# Autodesk Inventor assembly: chain(e)
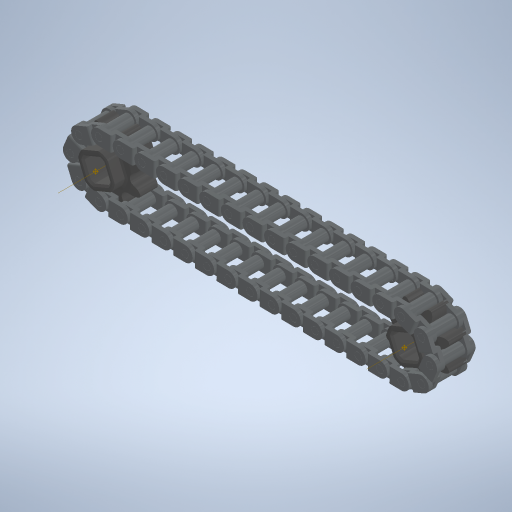
[picture p0: Inventor's stored thumbnail of the model, 512x512]
Saved by Autodesk Inventor 2023 (Build 270158000, 158)
## iProperties
Created: 2022-08-09
Part Number: chain(e)
Document SubType Name: Assembly
Designer: aaron
Author: aaron
## Documents named in this file (3)
- C:\Users\aaron\Documents\Inventor\Spin Up\library\Motion\New Sprockets\chain(e).iam
- C:\Users\aaron\Documents\Inventor\Spin Up\library\Motion\New Sprockets\8T.ipt
- C:\Users\aaron\Documents\Inventor\Spin Up\library\Motion\New Sprockets\IQ chain.ipt
## Components (38 placed, 2 different names)
1. 8T:1 — Mate:1, Mate:68, Mate:69, Mate:70, Mate:71, Flush:62, Mate:73
2. 8T:2 — Mate:1, Mate:63, Mate:64, Mate:65, Mate:66, Mate:67
3. IQ chain:12 — Mate:72, Mate:73
4. IQ chain:13
5. IQ chain:14
6. IQ chain:15
7. IQ chain:16 — Mate:31, Flush:30
8. IQ chain:17 — Mate:31, Flush:30
9. IQ chain:18
10. IQ chain:19
11. IQ chain:20
12. IQ chain:21
13. IQ chain:22
14. IQ chain:23
15. IQ chain:24
16. IQ chain:25
17. IQ chain:26 — Mate:63
18. IQ chain:27 — Mate:64
19. IQ chain:28 — Mate:65
20. IQ chain:29 — Mate:66
21. IQ chain:30 — Mate:67
22. IQ chain:31 — Mate:62, Flush:61
23. IQ chain:32 — Mate:62, Flush:61
24. IQ chain:33
25. IQ chain:34
26. IQ chain:35
27. IQ chain:36
28. IQ chain:37
29. IQ chain:38
30. IQ chain:39
31. IQ chain:40
32. IQ chain:41
33. IQ chain:42
34. IQ chain:43
35. IQ chain:44 — Mate:68
36. IQ chain:45 — Mate:69
37. IQ chain:46 — Mate:70
38. IQ chain:47 — Mate:71, Mate:72, Flush:62
## Relationships (83: Mate 47, Flush 36)
- Mate:1 (88.9 mm): 8T:1 ↔ 8T:2
- [Mate]: IQ chain:13 ↔ IQ chain:14
- [Flush]: IQ chain:13 ↔ IQ chain:14
- [Mate]: IQ chain:15 ↔ IQ chain:16
- [Flush]: IQ chain:15 ↔ IQ chain:16
- [Mate]: IQ chain:14 ↔ IQ chain:15
- [Flush]: IQ chain:14 ↔ IQ chain:15
- [Mate]: IQ chain:12 ↔ IQ chain:13
- [Flush]: IQ chain:12 ↔ IQ chain:13
- [Mate]: IQ chain:18 ↔ IQ chain:19
- [Flush]: IQ chain:18 ↔ IQ chain:19
- [Mate]: IQ chain:17 ↔ IQ chain:18
- [Flush]: IQ chain:17 ↔ IQ chain:18
- [Mate]: IQ chain:20 ↔ IQ chain:21
- [Flush]: IQ chain:20 ↔ IQ chain:21
- [Mate]: IQ chain:22 ↔ IQ chain:23
- [Flush]: IQ chain:22 ↔ IQ chain:23
- [Mate]: IQ chain:21 ↔ IQ chain:22
- [Flush]: IQ chain:21 ↔ IQ chain:22
- [Mate]: IQ chain:19 ↔ IQ chain:20
- [Flush]: IQ chain:19 ↔ IQ chain:20
- [Mate]: IQ chain:24 ↔ IQ chain:25
- [Flush]: IQ chain:24 ↔ IQ chain:25
- [Mate]: IQ chain:26 ↔ IQ chain:27
- [Flush]: IQ chain:26 ↔ IQ chain:27
- [Mate]: IQ chain:25 ↔ IQ chain:26
- [Flush]: IQ chain:25 ↔ IQ chain:26
- [Mate]: IQ chain:28 ↔ IQ chain:29
- [Flush]: IQ chain:28 ↔ IQ chain:29
- [Mate]: IQ chain:30 ↔ IQ chain:31
- [Flush]: IQ chain:30 ↔ IQ chain:31
- [Mate]: IQ chain:29 ↔ IQ chain:30
- [Flush]: IQ chain:29 ↔ IQ chain:30
- [Mate]: IQ chain:27 ↔ IQ chain:28
- [Flush]: IQ chain:27 ↔ IQ chain:28
- [Mate]: IQ chain:23 ↔ IQ chain:24
- [Flush]: IQ chain:23 ↔ IQ chain:24
- Mate:31: IQ chain:16 ↔ IQ chain:17
- Flush:30: IQ chain:16 ↔ IQ chain:17
- [Mate]: IQ chain:32 ↔ IQ chain:33
- [Flush]: IQ chain:32 ↔ IQ chain:33
- [Mate]: IQ chain:34 ↔ IQ chain:35
- [Flush]: IQ chain:34 ↔ IQ chain:35
- [Mate]: IQ chain:33 ↔ IQ chain:34
- [Flush]: IQ chain:33 ↔ IQ chain:34
- [Mate]: IQ chain:36 ↔ IQ chain:37
- [Flush]: IQ chain:36 ↔ IQ chain:37
- [Mate]: IQ chain:38 ↔ IQ chain:39
- [Flush]: IQ chain:38 ↔ IQ chain:39
- [Mate]: IQ chain:37 ↔ IQ chain:38
- [Flush]: IQ chain:37 ↔ IQ chain:38
- [Mate]: IQ chain:35 ↔ IQ chain:36
- [Flush]: IQ chain:35 ↔ IQ chain:36
- [Mate]: IQ chain:40 ↔ IQ chain:41
- [Flush]: IQ chain:40 ↔ IQ chain:41
- [Mate]: IQ chain:42 ↔ IQ chain:43
- [Flush]: IQ chain:42 ↔ IQ chain:43
- [Mate]: IQ chain:41 ↔ IQ chain:42
- [Flush]: IQ chain:41 ↔ IQ chain:42
- [Mate]: IQ chain:44 ↔ IQ chain:45
- [Flush]: IQ chain:44 ↔ IQ chain:45
- [Mate]: IQ chain:46 ↔ IQ chain:47
- [Flush]: IQ chain:46 ↔ IQ chain:47
- [Mate]: IQ chain:45 ↔ IQ chain:46
- [Flush]: IQ chain:45 ↔ IQ chain:46
- [Mate]: IQ chain:43 ↔ IQ chain:44
- [Flush]: IQ chain:43 ↔ IQ chain:44
- [Mate]: IQ chain:39 ↔ IQ chain:40
- [Flush]: IQ chain:39 ↔ IQ chain:40
- Mate:62: IQ chain:31 ↔ IQ chain:32
- Flush:61: IQ chain:31 ↔ IQ chain:32
- Mate:63: 8T:2 ↔ IQ chain:26
- Mate:64: 8T:2 ↔ IQ chain:27
- Mate:65: 8T:2 ↔ IQ chain:28
- Mate:66: 8T:2 ↔ IQ chain:29
- Mate:67: 8T:2 ↔ IQ chain:30
- Mate:68: 8T:1 ↔ IQ chain:44
- Mate:69: 8T:1 ↔ IQ chain:45
- Mate:70: 8T:1 ↔ IQ chain:46
- Mate:71: 8T:1 ↔ IQ chain:47
- Mate:72: IQ chain:12 ↔ IQ chain:47
- Flush:62 (-0.762 mm): 8T:1 ↔ IQ chain:47
- Mate:73: 8T:1 ↔ IQ chain:12
## Named parameters: d19_d7_d3_d1 = 0 mm, d20_d8_d4_d2 = 0 mm, d21_d9_d5 = 0 mm, d22_d10_d6 = 0 mm, d23_d11_d1 = 0 mm, d24_d12_d2 = 0 mm, d25_d13 = 0 mm, d26_d14 = 0 mm, d31_d3_d1 = 0 mm, d32_d4_d2 = 0 mm, d33_d5 = 0 mm, d34_d6 = 0 mm, d35_d7_d3_d1 = 0 mm, d36_d8_d4_d2 = 0 mm, d37_d9_d5 = 0 mm, d38_d10_d6 = 0 mm, d39_d11_d1 = 0 mm, d40_d12_d2 = 0 mm, d41_d13 = 0 mm, d42_d14 = 0 mm, d43_d15_d3_d1 = 0 mm, d44_d16_d4_d2 = 0 mm, d45_d17_d5 = 0 mm, d46_d18_d6 = 0 mm, d47_d19_d7_d3_d1 = 0 mm, d48_d20_d8_d4_d2 = 0 mm, d49_d21_d9_d5 = 0 mm, d50_d22_d10_d6 = 0 mm, d51_d23_d11_d1 = 0 mm, d52_d24_d12_d2 = 0 mm, d53_d25_d13 = 0 mm, d54_d26_d14 = 0 mm, d55_d27_d1 = 0 mm, d56_d28_d2 = 0 mm, d57_d29 = 0 mm, d58_d30 = 0 mm, d68_d3_d1 = 0 mm, d69_d4_d2 = 0 mm, d70_d5 = 0 mm, d71_d6 = 0 mm, d72_d7_d3_d1 = 0 mm, d73_d8_d4_d2 = 0 mm, d74_d9_d5 = 0 mm, d75_d10_d6 = 0 mm, d76_d11_d1 = 0 mm, d77_d12_d2 = 0 mm, d78_d13 = 0 mm, d79_d14 = 0 mm, d80_d15_d3_d1 = 0 mm, d81_d16_d4_d2 = 0 mm, d82_d17_d5 = 0 mm, d83_d18_d6 = 0 mm, d84_d19_d7_d3_d1 = 0 mm, d85_d20_d8_d4_d2 = 0 mm, d86_d21_d9_d5 = 0 mm, d87_d22_d10_d6 = 0 mm, d88_d23_d11_d1 = 0 mm, d89_d24_d12_d2 = 0 mm, d90_d25_d13 = 0 mm, d91_d26_d14 = 0 mm, d92_d27_d1 = 0 mm, d93_d28_d2 = 0 mm, d94_d29 = 0 mm, d95_d30 = 0 mm, d119_d1 = 0 mm, d120_d2 = 0 mm
